# Autodesk Inventor assembly: Assembly1
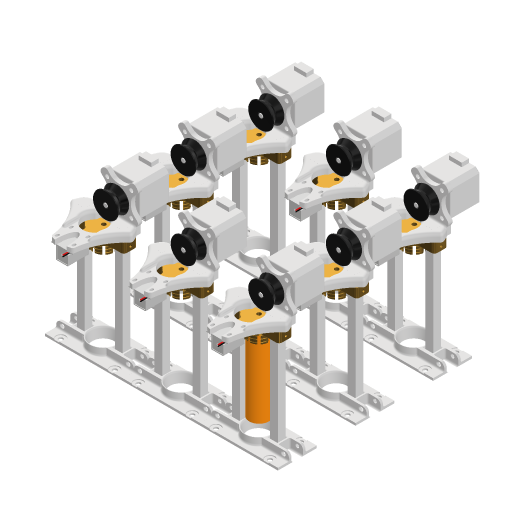
[picture p0: Inventor's stored thumbnail of the model, 512x512]
Saved by Autodesk Inventor 2023 (Build 270158000, 158)
## iProperties
Created: 2022-10-31
Part Number: Assembly1
Document SubType Name: Assembly
Designer: Dave
Author: Dave
## Documents named in this file (4)
- C:\GrabCAD\Chalk Bot\Chalkbot1.0\Apparatus\V5\8Pc Base Assembly.iam
- C:\GrabCAD\Chalk Bot\Chalkbot1.0\Apparatus\V5\Base.ipt
- C:\GrabCAD\Chalk Bot\Chalkbot1.0\Apparatus\V5\ApparatusMasterAssemV5.iam
- C:\GrabCAD\Chalk Bot\Chalkbot1.0\Apparatus\V5\Chalk.ipt
## Components (18 placed, 3 different names)
1. Chalk:1 — Mate:4
2. Base:1
3. Base:2
4. Base:3
5. Base:4
6. Base:5
7. Base:6
8. Base:7
9. Base:8 — Mate:3
10. Base:9 — Mate:1, Mate:2
11. ApparatusMasterAssemV5:1 [sub-assembly] — Mate:1, Mate:2, Mate:3, Mate:4
12. ApparatusMasterAssemV5:2 [sub-assembly]
13. ApparatusMasterAssemV5:3 [sub-assembly]
14. ApparatusMasterAssemV5:4 [sub-assembly]
15. ApparatusMasterAssemV5:6 [sub-assembly]
16. ApparatusMasterAssemV5:7 [sub-assembly]
17. ApparatusMasterAssemV5:8 [sub-assembly]
18. ApparatusMasterAssemV5:9 [sub-assembly]
## Component patterns: (9 elements, first: Base:1), (9 elements, first: ApparatusMasterAssemV5:1)
## Relationships (4: Mate 4)
- Mate:1: Base:9 ↔ ApparatusMasterAssemV5:1
- Mate:2: Base:9 ↔ ApparatusMasterAssemV5:1
- Mate:3: Base:8 ↔ ApparatusMasterAssemV5:1
- Mate:4: Chalk:1 ↔ ApparatusMasterAssemV5:1
